# Autodesk Inventor assembly: slidebox
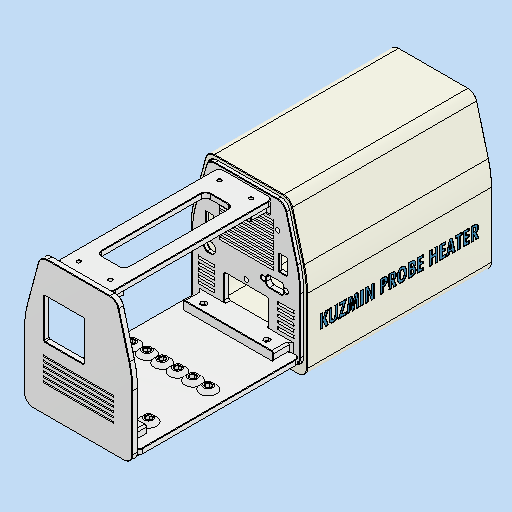
[picture p0: Inventor's stored thumbnail of the model, 512x512]
Saved by Autodesk Inventor 2026 (Build 300175050, 175E)
## iProperties
Created: 2025-06-12
Part Number: slidebox
Document SubType Name: Assembly
Designer: queezz
Author: queezz
## Documents named in this file (6)
- C:\Users\queezz\Dropbox\Drawings\PIHTI\ElectronicsBox\slidebox-teplate\slidebox.iam
- C:\Users\queezz\Dropbox\Drawings\PIHTI\ElectronicsBox\slidebox-teplate\slidebox-back-panel.ipt
- C:\Users\queezz\Dropbox\Drawings\PIHTI\ElectronicsBox\slidebox-teplate\slidebox-bottom-tray.ipt
- C:\Users\queezz\Dropbox\Drawings\PIHTI\ElectronicsBox\slidebox-teplate\slidebox-case.ipt
- C:\Users\queezz\Dropbox\Drawings\PIHTI\ElectronicsBox\slidebox-teplate\slidebox-front-panel.ipt
- C:\Users\queezz\Dropbox\Drawings\PIHTI\ElectronicsBox\slidebox-teplate\slidebox-top-bar.ipt
## Components (5 placed, 5 different names)
1. slidebox-back-panel:1 — Rigid:2, Rigid:3
2. slidebox-bottom-tray:1 — Rigid:3, Flush:3
3. slidebox-case:1 — Flush:4, Flush:5
4. slidebox-front-panel:1 — Rigid:1, Flush:1, Flush:2, Flush:5
5. slidebox-top-bar:1 — Rigid:1, Rigid:2
## Relationships (8: Flush 5, WeldJoint 3)
- Rigid:1 [WeldJoint]: slidebox-front-panel:1 ↔ slidebox-top-bar:1
- Rigid:2 [WeldJoint]: slidebox-back-panel:1 ↔ slidebox-top-bar:1
- Rigid:3 [WeldJoint]: slidebox-back-panel:1 ↔ slidebox-bottom-tray:1
- Flush:1: slidebox-front-panel:1
- Flush:2: slidebox-front-panel:1
- Flush:3: slidebox-bottom-tray:1
- Flush:4: slidebox-case:1
- Flush:5: slidebox-case:1 ↔ slidebox-front-panel:1
